# Autodesk Inventor assembly: robot4
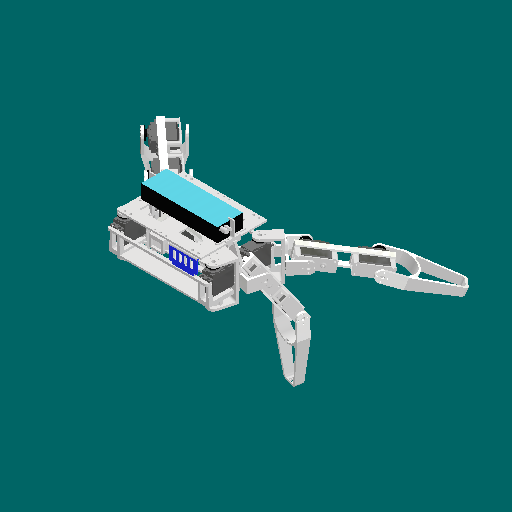
[picture p0: Inventor's stored thumbnail of the model, 512x512]
Saved by Autodesk Inventor 2026.1 (Build 301233000, 233)
## iProperties
Created: 2025-11-03
Part Number: robot4
Document SubType Name: Assembly
Designer: emanuel
Author: emanuel
## Documents named in this file (18)
- C:\Users\emanuel\UnFolder\SpiderRobo\3dmodel\robot4.iam
- C:\Users\emanuel\UnFolder\SpiderRobo\3dmodel\rigid_support1.ipt
- C:\Users\emanuel\UnFolder\SpiderRobo\3dmodel\support_2_servos.ipt
- C:\Users\emanuel\UnFolder\SpiderRobo\3dmodel\mg996r.ipt
- C:\Users\emanuel\UnFolder\SpiderRobo\3dmodel\servo_support_4.ipt
- C:\Users\emanuel\UnFolder\SpiderRobo\3dmodel\rigid_support3.ipt
- C:\Users\emanuel\UnFolder\SpiderRobo\3dmodel\servo_disc.ipt
- C:\Users\emanuel\UnFolder\SpiderRobo\3dmodel\C1.ipt
- C:\Users\emanuel\UnFolder\SpiderRobo\3dmodel\battery1.ipt
- C:\Users\emanuel\UnFolder\SpiderRobo\3dmodel\back_plate.ipt
- C:\Users\emanuel\UnFolder\SpiderRobo\3dmodel\smart_calf.ipt
- C:\Users\emanuel\UnFolder\SpiderRobo\3dmodel\back_servo_support.ipt
- C:\Users\emanuel\UnFolder\SpiderRobo\3dmodel\C2.ipt
- C:\Users\emanuel\UnFolder\SpiderRobo\3dmodel\femur.ipt
- C:\Users\emanuel\UnFolder\SpiderRobo\3dmodel\rigid_support2.ipt
- C:\Users\emanuel\UnFolder\SpiderRobo\3dmodel\power_button_holder.ipt
- C:\Users\emanuel\UnFolder\SpiderRobo\3dmodel\battery_holder_1.ipt
- C:\Users\emanuel\UnFolder\SpiderRobo\3dmodel\lateral_panel_1.ipt
## Components (86 placed, 17 different names)
1. rigid_support1:1 — Mate:47, Mate:48, Flush:7, Flush:8, Flush:9
2. rigid_support1:2 — Flush:7, Flush:10, Flush:11, Mate:49, Flush:12, Flush:13
3. support_2_servos:3 — Mate:17, Mate:18, Mate:19, Mate:48, Mate:49, Flush:12, Flush:13, Mate:252, Flush:14, Flush:15
4. mg996r:1 — Mate:7, Mate:8, Mate:20, Mate:21, Mate:63, Mate:64, Mate:251, Mate:253
5. servo_support_4:3 — Flush:1, Flush:3
6. servo_support_4:4 — Flush:1, Mate:7, Mate:8, Mate:252, Flush:14, Flush:15, Mate:263
7. mg996r:2 — Mate:22, Mate:23, Mate:254, Mate:255, Mate:257
8. servo_support_4:5 — Mate:62
9. servo_support_4:6 — Flush:3, Mate:17, Mate:18, Mate:19, Mate:258, Mate:259, Mate:260
10. servo_disc:1 — Mate:20, Mate:21, Mate:250
11. servo_disc:2 — Mate:22, Mate:23, Mate:256
12. support_2_servos:4 — Mate:47, Flush:8, Flush:9, Flush:10, Flush:11
13. mg996r:3 — Mate:247
14. servo_support_4:7
15. servo_support_4:8 — Mate:261, Mate:262
16. rigid_support3:2 — Mate:66, Mate:67
17. mg996r:4 — Mate:249
18. servo_support_4:9
19. servo_support_4:10
20. servo_disc:3 — Mate:246
21. servo_disc:4 — Mate:248
22. rigid_support3:3 — Mate:62, Mate:63, Mate:64, Mate:65, Mate:253, Mate:254, Mate:255
23. back_plate:1 — Mate:65, Mate:66, Mate:67, Mate:264, Mate:265, Mate:266, Mate:267, Mate:268, Mate:269, Mate:270, Mate:271, Mate:272, Mate:273, Mate:276, Mate:277, Mate:278
24. smart_calf:1 — Mate:128, Mate:129
25. servo_disc:7 — Mate:128
26. back_servo_support:3
27. C2:2 — Mate:130, Mate:131, Mate:132, Mate:133, Mate:134
28. femur:2
29. mg996r:7 — Mate:129
30. servo_disc:8
31. mg996r:8
32. back_servo_support:4
33. servo_support_4:16
34. servo_support_4:17
35. servo_support_4:18
36. servo_support_4:19
37. C1:1 — Mate:130, Mate:131, Mate:132, Mate:133, Mate:134, Mate:248, Mate:249
38. smart_calf:2
39. servo_disc:9
40. back_servo_support:5
41. C2:3
42. femur:3
43. mg996r:9
44. servo_disc:10
45. mg996r:10
46. back_servo_support:6
47. servo_support_4:20
48. servo_support_4:21
49. servo_support_4:22
50. servo_support_4:23
51. C1:2 — Mate:256, Mate:257
52. smart_calf:3
53. servo_disc:11
54. back_servo_support:7
55. C2:4
56. femur:4
57. mg996r:11
58. servo_disc:12
59. mg996r:12
60. back_servo_support:8
61. servo_support_4:24
62. servo_support_4:25
63. servo_support_4:26
64. servo_support_4:27
65. C1:3 — Mate:250, Mate:251
66. smart_calf:4
67. servo_disc:13
68. back_servo_support:9
69. C2:5
70. femur:5
71. mg996r:13
72. servo_disc:14
73. mg996r:14
74. back_servo_support:10
75. servo_support_4:28
76. servo_support_4:29
77. servo_support_4:30
78. servo_support_4:31
79. C1:4 — Mate:246, Mate:247
80. rigid_support2:1 — Mate:258, Mate:259, Mate:260
81. rigid_support2:2 — Mate:261, Mate:262, Mate:263
82. power_button_holder:1 — Mate:264, Mate:265, Mate:266
83. battery1:1 — Mate:267, Mate:274, Mate:275
84. battery_holder_1:1 — Mate:271, Mate:272, Mate:273, Mate:274
85. battery_holder_1:2 — Mate:268, Mate:269, Mate:270, Mate:275
86. lateral_panel_1:1 — Mate:276, Mate:277, Mate:278
## Relationships (239: Mate 224, Flush 15)
- Flush:1: servo_support_4:3 ↔ servo_support_4:4
- Mate:7: mg996r:1 ↔ servo_support_4:4
- Mate:8: mg996r:1 ↔ servo_support_4:4
- [Flush]: servo_support_4:5 ↔ servo_support_4:6
- [Mate]: mg996r:2 ↔ servo_support_4:6
- [Mate]: mg996r:2 ↔ servo_support_4:6
- Flush:3: servo_support_4:3 ↔ servo_support_4:6
- Mate:17: support_2_servos:3 ↔ servo_support_4:6
- Mate:18: support_2_servos:3 ↔ servo_support_4:6
- Mate:19: support_2_servos:3 ↔ servo_support_4:6
- Mate:20: mg996r:1 ↔ servo_disc:1
- Mate:21: mg996r:1 ↔ servo_disc:1
- Mate:22: mg996r:2 ↔ servo_disc:2
- Mate:23: mg996r:2 ↔ servo_disc:2
- [Mate]: mg996r:3 ↔ rigid_support3:2
- [Mate]: mg996r:3 ↔ rigid_support3:2
- [Mate]: mg996r:3 ↔ rigid_support3:2
- [Mate]: servo_support_4:7 ↔ rigid_support3:2
- [Flush]: servo_support_4:7 ↔ servo_support_4:8
- [Mate]: servo_support_4:7 ↔ rigid_support3:2
- [Mate]: servo_support_4:7 ↔ rigid_support3:2
- [Mate]: mg996r:3 ↔ servo_support_4:8
- [Mate]: mg996r:3 ↔ servo_support_4:8
- [Flush]: servo_support_4:9 ↔ servo_support_4:10
- [Mate]: mg996r:4 ↔ servo_support_4:10
- [Mate]: mg996r:4 ↔ servo_support_4:10
- [Mate]: rigid_support3:2 ↔ servo_support_4:9
- [Mate]: rigid_support3:2 ↔ servo_support_4:9
- [Mate]: rigid_support3:2 ↔ servo_support_4:9
- [Mate]: rigid_support3:2 ↔ mg996r:4
- [Mate]: rigid_support3:2 ↔ mg996r:4
- [Mate]: rigid_support3:2 ↔ mg996r:4
- [Flush]: servo_support_4:7 ↔ servo_support_4:10
- [Mate]: support_2_servos:4 ↔ servo_support_4:10
- [Mate]: support_2_servos:4 ↔ servo_support_4:10
- [Mate]: support_2_servos:4 ↔ servo_support_4:10
- [Mate]: mg996r:3 ↔ servo_disc:3
- [Mate]: mg996r:3 ↔ servo_disc:3
- [Mate]: mg996r:4 ↔ servo_disc:4
- [Mate]: mg996r:4 ↔ servo_disc:4
- Mate:47: rigid_support1:1 ↔ support_2_servos:4
- Mate:48: rigid_support1:1 ↔ support_2_servos:3
- Flush:7: rigid_support1:1 ↔ rigid_support1:2
- Flush:8: rigid_support1:1 ↔ support_2_servos:4
- Flush:9: rigid_support1:1 ↔ support_2_servos:4
- Flush:10: rigid_support1:2 ↔ support_2_servos:4
- Flush:11: rigid_support1:2 ↔ support_2_servos:4
- Mate:49: rigid_support1:2 ↔ support_2_servos:3
- Flush:12: rigid_support1:2 ↔ support_2_servos:3
- Flush:13: rigid_support1:2 ↔ support_2_servos:3
- Mate:62: servo_support_4:5 ↔ rigid_support3:3
- Mate:63: mg996r:1 ↔ rigid_support3:3
- Mate:64: mg996r:1 ↔ rigid_support3:3
- Mate:65: rigid_support3:3 ↔ back_plate:1
- Mate:66: rigid_support3:2 ↔ back_plate:1
- Mate:67: rigid_support3:2 ↔ back_plate:1
- [Mate]: servo_disc:7 ↔ mg996r:7
- [Mate]: servo_disc:7 ↔ mg996r:7
- [Mate]: servo_disc:8 ↔ mg996r:8
- [Mate]: servo_disc:8 ↔ mg996r:8
- [Mate]: femur:2 ↔ mg996r:8
- [Mate]: femur:2 ↔ mg996r:8
- [Mate]: femur:2 ↔ mg996r:8
- [Mate]: femur:2 ↔ mg996r:7
- [Mate]: femur:2 ↔ mg996r:7
- [Mate]: femur:2 ↔ mg996r:7
- [Mate]: C2:2 ↔ servo_disc:8
- [Mate]: C2:2 ↔ mg996r:8
- [Mate]: femur:2 ↔ servo_support_4:16
- [Mate]: femur:2 ↔ servo_support_4:19
- [Mate]: femur:2 ↔ servo_support_4:17
- [Mate]: femur:2 ↔ servo_support_4:18
- [Mate]: femur:2 ↔ servo_support_4:16
- [Mate]: mg996r:7 ↔ servo_support_4:19
- [Mate]: back_servo_support:4 ↔ servo_support_4:16
- [Mate]: back_servo_support:4 ↔ servo_support_4:16
- [Mate]: back_servo_support:4 ↔ servo_support_4:16
- [Mate]: back_servo_support:4 ↔ servo_support_4:19
- [Mate]: femur:2 ↔ servo_support_4:16
- [Mate]: femur:2 ↔ servo_support_4:18
- [Mate]: femur:2 ↔ servo_support_4:18
- [Mate]: mg996r:8 ↔ servo_support_4:17
- [Mate]: back_servo_support:3 ↔ servo_support_4:18
- [Mate]: back_servo_support:3 ↔ servo_support_4:18
- [Mate]: back_servo_support:3 ↔ servo_support_4:18
- [Mate]: back_servo_support:3 ↔ servo_support_4:17
- Mate:128: smart_calf:1 ↔ servo_disc:7
- Mate:129: smart_calf:1 ↔ mg996r:7
- Mate:130: C2:2 ↔ C1:1
- Mate:131: C2:2 ↔ C1:1
- Mate:132: C2:2 ↔ C1:1
- Mate:133: C2:2 ↔ C1:1
- Mate:134: C2:2 ↔ C1:1
- [Mate]: servo_disc:9 ↔ mg996r:9
- [Mate]: servo_disc:9 ↔ mg996r:9
- [Mate]: servo_disc:10 ↔ mg996r:10
- [Mate]: servo_disc:10 ↔ mg996r:10
- [Mate]: femur:3 ↔ mg996r:10
- [Mate]: femur:3 ↔ mg996r:10
- [Mate]: femur:3 ↔ mg996r:10
- [Mate]: femur:3 ↔ mg996r:9
- [Mate]: femur:3 ↔ mg996r:9
- [Mate]: femur:3 ↔ mg996r:9
- [Mate]: C2:3 ↔ servo_disc:10
- [Mate]: C2:3 ↔ mg996r:10
- [Mate]: femur:3 ↔ servo_support_4:20
- [Mate]: femur:3 ↔ servo_support_4:23
- [Mate]: femur:3 ↔ servo_support_4:21
- [Mate]: femur:3 ↔ servo_support_4:22
- [Mate]: femur:3 ↔ servo_support_4:20
- [Mate]: mg996r:9 ↔ servo_support_4:23
- [Mate]: back_servo_support:6 ↔ servo_support_4:20
- [Mate]: back_servo_support:6 ↔ servo_support_4:20
- [Mate]: back_servo_support:6 ↔ servo_support_4:20
- [Mate]: back_servo_support:6 ↔ servo_support_4:23
- [Mate]: femur:3 ↔ servo_support_4:20
- [Mate]: femur:3 ↔ servo_support_4:22
- [Mate]: femur:3 ↔ servo_support_4:22
- [Mate]: mg996r:10 ↔ servo_support_4:21
- [Mate]: back_servo_support:5 ↔ servo_support_4:22
- [Mate]: back_servo_support:5 ↔ servo_support_4:22
- [Mate]: back_servo_support:5 ↔ servo_support_4:22
- [Mate]: back_servo_support:5 ↔ servo_support_4:21
- [Mate]: smart_calf:2 ↔ servo_disc:9
- [Mate]: smart_calf:2 ↔ mg996r:9
- [Mate]: C2:3 ↔ C1:2
- [Mate]: C2:3 ↔ C1:2
- [Mate]: C2:3 ↔ C1:2
- [Mate]: C2:3 ↔ C1:2
- [Mate]: C2:3 ↔ C1:2
- [Mate]: servo_disc:11 ↔ mg996r:11
- [Mate]: servo_disc:11 ↔ mg996r:11
- [Mate]: servo_disc:12 ↔ mg996r:12
- [Mate]: servo_disc:12 ↔ mg996r:12
- [Mate]: femur:4 ↔ mg996r:12
- [Mate]: femur:4 ↔ mg996r:12
- [Mate]: femur:4 ↔ mg996r:12
- [Mate]: femur:4 ↔ mg996r:11
- [Mate]: femur:4 ↔ mg996r:11
- [Mate]: femur:4 ↔ mg996r:11
- [Mate]: C2:4 ↔ servo_disc:12
- [Mate]: C2:4 ↔ mg996r:12
- [Mate]: femur:4 ↔ servo_support_4:24
- [Mate]: femur:4 ↔ servo_support_4:27
- [Mate]: femur:4 ↔ servo_support_4:25
- [Mate]: femur:4 ↔ servo_support_4:26
- [Mate]: femur:4 ↔ servo_support_4:24
- [Mate]: mg996r:11 ↔ servo_support_4:27
- [Mate]: back_servo_support:8 ↔ servo_support_4:24
- [Mate]: back_servo_support:8 ↔ servo_support_4:24
- [Mate]: back_servo_support:8 ↔ servo_support_4:24
- [Mate]: back_servo_support:8 ↔ servo_support_4:27
- [Mate]: femur:4 ↔ servo_support_4:24
- [Mate]: femur:4 ↔ servo_support_4:26
- [Mate]: femur:4 ↔ servo_support_4:26
- [Mate]: mg996r:12 ↔ servo_support_4:25
- [Mate]: back_servo_support:7 ↔ servo_support_4:26
- [Mate]: back_servo_support:7 ↔ servo_support_4:26
- [Mate]: back_servo_support:7 ↔ servo_support_4:26
- [Mate]: back_servo_support:7 ↔ servo_support_4:25
- [Mate]: smart_calf:3 ↔ servo_disc:11
- [Mate]: smart_calf:3 ↔ mg996r:11
- [Mate]: C2:4 ↔ C1:3
- [Mate]: C2:4 ↔ C1:3
- [Mate]: C2:4 ↔ C1:3
- [Mate]: C2:4 ↔ C1:3
- [Mate]: C2:4 ↔ C1:3
- [Mate]: servo_disc:13 ↔ mg996r:13
- [Mate]: servo_disc:13 ↔ mg996r:13
- [Mate]: servo_disc:14 ↔ mg996r:14
- [Mate]: servo_disc:14 ↔ mg996r:14
- [Mate]: femur:5 ↔ mg996r:14
- [Mate]: femur:5 ↔ mg996r:14
- [Mate]: femur:5 ↔ mg996r:14
- [Mate]: femur:5 ↔ mg996r:13
- [Mate]: femur:5 ↔ mg996r:13
- [Mate]: femur:5 ↔ mg996r:13
- [Mate]: C2:5 ↔ servo_disc:14
- [Mate]: C2:5 ↔ mg996r:14
- [Mate]: femur:5 ↔ servo_support_4:28
- [Mate]: femur:5 ↔ servo_support_4:31
- [Mate]: femur:5 ↔ servo_support_4:29
- [Mate]: femur:5 ↔ servo_support_4:30
- [Mate]: femur:5 ↔ servo_support_4:28
- [Mate]: mg996r:13 ↔ servo_support_4:31
- [Mate]: back_servo_support:10 ↔ servo_support_4:28
- [Mate]: back_servo_support:10 ↔ servo_support_4:28
- [Mate]: back_servo_support:10 ↔ servo_support_4:28
- [Mate]: back_servo_support:10 ↔ servo_support_4:31
- [Mate]: femur:5 ↔ servo_support_4:28
- [Mate]: femur:5 ↔ servo_support_4:30
- [Mate]: femur:5 ↔ servo_support_4:30
- [Mate]: mg996r:14 ↔ servo_support_4:29
- [Mate]: back_servo_support:9 ↔ servo_support_4:30
- [Mate]: back_servo_support:9 ↔ servo_support_4:30
- [Mate]: back_servo_support:9 ↔ servo_support_4:30
- [Mate]: back_servo_support:9 ↔ servo_support_4:29
- [Mate]: smart_calf:4 ↔ servo_disc:13
- [Mate]: smart_calf:4 ↔ mg996r:13
- [Mate]: C2:5 ↔ C1:4
- [Mate]: C2:5 ↔ C1:4
- [Mate]: C2:5 ↔ C1:4
- [Mate]: C2:5 ↔ C1:4
- [Mate]: C2:5 ↔ C1:4
- Mate:246: servo_disc:3 ↔ C1:4
- Mate:247: mg996r:3 ↔ C1:4
- Mate:248: servo_disc:4 ↔ C1:1
- Mate:249: mg996r:4 ↔ C1:1
- Mate:250: servo_disc:1 ↔ C1:3
- Mate:251: mg996r:1 ↔ C1:3
- Mate:252: support_2_servos:3 ↔ servo_support_4:4
- Flush:14: support_2_servos:3 ↔ servo_support_4:4
- Flush:15: support_2_servos:3 ↔ servo_support_4:4
- Mate:253: mg996r:1 ↔ rigid_support3:3
- Mate:254: mg996r:2 ↔ rigid_support3:3
- Mate:255: mg996r:2 ↔ rigid_support3:3
- Mate:256: servo_disc:2 ↔ C1:2
- Mate:257: mg996r:2 ↔ C1:2
- Mate:258: servo_support_4:6 ↔ rigid_support2:1
- Mate:259: servo_support_4:6 ↔ rigid_support2:1
- Mate:260: servo_support_4:6 ↔ rigid_support2:1
- Mate:261: servo_support_4:8 ↔ rigid_support2:2
- Mate:262: servo_support_4:8 ↔ rigid_support2:2
- Mate:263: servo_support_4:4 ↔ rigid_support2:2
- Mate:264: back_plate:1 ↔ power_button_holder:1
- Mate:265: back_plate:1 ↔ power_button_holder:1
- Mate:266: back_plate:1 ↔ power_button_holder:1
- Mate:267: back_plate:1 ↔ battery1:1
- Mate:268: back_plate:1 ↔ battery_holder_1:2
- Mate:269: back_plate:1 ↔ battery_holder_1:2
- Mate:270: back_plate:1 ↔ battery_holder_1:2
- Mate:271: back_plate:1 ↔ battery_holder_1:1
- Mate:272: back_plate:1 ↔ battery_holder_1:1
- Mate:273: back_plate:1 ↔ battery_holder_1:1
- Mate:274: battery1:1 ↔ battery_holder_1:1
- Mate:275: battery1:1 ↔ battery_holder_1:2
- Mate:276: back_plate:1 ↔ lateral_panel_1:1
- Mate:277: back_plate:1 ↔ lateral_panel_1:1
- Mate:278: back_plate:1 ↔ lateral_panel_1:1
## Named parameters: d24_d19 = 0 mm, d25_d22 = 0 mm, d26_d23 = 0 mm, d41_d15 = 0 mm, d42_d16 = 0 mm, d43_d17 = 0 mm, d44_d18 = 0 mm, d45_d19 = 0 mm, d46_d20 = 0 mm, d47_d21 = 0 mm, d48_d22 = 0 mm, d49_d23 = 0 mm, d50_d24_d19 = 0 mm, d51_d25_d22 = 0 mm, d52_d26_d23 = 0 mm, d53_d27 = 0 mm, d54_d28 = 0 mm, d55_d29 = 0 mm, d56_d30 = 0 mm, d57_d31 = 0 mm, d58_d32 = 0 mm, d59_d33 = 0 mm, d60_d34 = 0 mm, d61_d35 = 0 mm, d62_d36 = 0 mm, d63_d37 = 0 mm, d64_d38 = 0 mm, d65_d39 = 0 mm, d66_d40 = 0 mm, d125_d101 = 0 mm, d126_d102 = 0 mm, d127_d103 = 0 mm, d128_d104 = 0 mm, d129_d105 = 0 mm, d130_d106 = 0 mm, d131_d107 = 0 mm, d132_d108 = 0 mm, d133_d109 = 0 mm, d134_d110 = 0 mm, d135_d111 = 0 mm, d136_d112 = 0 mm, d137_d113 = 0 mm, d138_d114 = 0 mm, d139_d115 = 0 mm, d140_d116 = 0 mm, d141_d117 = 0 mm, d142_d118 = 0 mm, d143_d119 = 0 mm, d144_d120 = 0 mm, d145_d121 = 0 mm, d146_d122 = 0 mm, d147_d123 = 0 mm, d148_d124 = 0 mm, d149_d95 = 0 mm, d150_d96 = 0 mm, d151_d97_d95 = 0 mm, d152_d98_d96 = 0 mm, d153_d99 = 0 mm, d154_d100 = 0 mm, d231_d226 = 0 mm, d232_d227 = 0 mm, d233_d228 = 0 mm, d234_d229 = 0 mm, d235_d155 = 0 mm, d236_d156 = 0 mm, d237_d125_d101 = 0 mm, d238_d126_d102 = 0 mm, d239_d127_d103 = 0 mm, d240_d128_d104 = 0 mm, d241_d129_d105 = 0 mm, d242_d130_d106 = 0 mm, d243_d131_d107 = 0 mm, d244_d132_d108 = 0 mm, d245_d133_d109 = 0 mm, d246_d134_d110 = 0 mm, d247_d135_d111 = 0 mm, d248_d136_d112 = 0 mm, d249_d137_d113 = 0 mm, d250_d138_d114 = 0 mm, d251_d139_d115 = 0 mm, d252_d140_d116 = 0 mm, d253_d141_d117 = 0 mm, d254_d142_d118 = 0 mm, d255_d143_d119 = 0 mm, d256_d144_d120 = 0 mm, d257_d145_d121 = 0 mm, d258_d146_d122 = 0 mm, d259_d147_d123 = 0 mm, d260_d148_d124 = 0 mm, d261_d149_d95 = 0 mm, d262_d150_d96 = 0 mm, d263_d151_d97_d95 = 0 mm, d264_d152_d98_d96 = 0 mm, d265_d153_d99 = 0 mm, d266_d154_d100 = 0 mm, d267_d230 = 0 mm, d268_d226 = 0 mm, d269_d227 = 0 mm, d270_d228 = 0 mm, d271_d229 = 0 mm, d272_d155 = 0 mm, d273_d156 = 0 mm, d274_d125_d101 = 0 mm, d275_d126_d102 = 0 mm, d276_d127_d103 = 0 mm, d277_d128_d104 = 0 mm, d278_d129_d105 = 0 mm, d279_d130_d106 = 0 mm, d280_d131_d107 = 0 mm, d281_d132_d108 = 0 mm, d282_d133_d109 = 0 mm, d283_d134_d110 = 0 mm, d284_d135_d111 = 0 mm, d285_d136_d112 = 0 mm, d286_d137_d113 = 0 mm, d287_d138_d114 = 0 mm, d288_d139_d115 = 0 mm, d289_d140_d116 = 0 mm, d290_d141_d117 = 0 mm, d291_d142_d118 = 0 mm, d292_d143_d119 = 0 mm, d293_d144_d120 = 0 mm, d294_d145_d121 = 0 mm, d295_d146_d122 = 0 mm, d296_d147_d123 = 0 mm, d297_d148_d124 = 0 mm, d298_d149_d95 = 0 mm, d299_d150_d96 = 0 mm, d300_d151_d97_d95 = 0 mm, d301_d152_d98_d96 = 0 mm, d302_d153_d99 = 0 mm, d303_d154_d100 = 0 mm, d304_d230 = 0 mm, d305_d226 = 0 mm, d306_d227 = 0 mm, d307_d228 = 0 mm, d308_d229 = 0 mm, d309_d155 = 0 mm, d310_d156 = 0 mm, d311_d125_d101 = 0 mm, d312_d126_d102 = 0 mm, d313_d127_d103 = 0 mm, d314_d128_d104 = 0 mm, d315_d129_d105 = 0 mm, d316_d130_d106 = 0 mm, d317_d131_d107 = 0 mm, d318_d132_d108 = 0 mm, d319_d133_d109 = 0 mm, d320_d134_d110 = 0 mm, d321_d135_d111 = 0 mm, d322_d136_d112 = 0 mm, d323_d137_d113 = 0 mm, d324_d138_d114 = 0 mm, d325_d139_d115 = 0 mm, d326_d140_d116 = 0 mm, d327_d141_d117 = 0 mm, d328_d142_d118 = 0 mm, d329_d143_d119 = 0 mm, d330_d144_d120 = 0 mm, d331_d145_d121 = 0 mm, d332_d146_d122 = 0 mm, d333_d147_d123 = 0 mm, d334_d148_d124 = 0 mm, d335_d149_d95 = 0 mm, d336_d150_d96 = 0 mm, d337_d151_d97_d95 = 0 mm, d338_d152_d98_d96 = 0 mm, d339_d153_d99 = 0 mm, d340_d154_d100 = 0 mm, d341_d230 = 0 mm
